# Autodesk Inventor assembly: centre wing
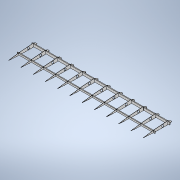
[picture p0: Inventor's stored thumbnail of the model, 180x180]
Saved by Autodesk Inventor 2021 (Build 250183000, 183)
## iProperties
Created: 2021-03-09
Part Number: centre wing
Document SubType Name: Assembly
Designer: Ferdinand Hubbard
Author: Ferdinand Hubbard
## Documents named in this file (4)
- C:\Users\Ferdinand Hubbard\Desktop\solarplane\cad\centre wing.iam
- C:\Users\Ferdinand Hubbard\Desktop\solarplane\cad\airfoil.ipt
- C:\Users\Ferdinand Hubbard\Desktop\solarplane\cad\centre back wood spar.ipt
- C:\Users\Ferdinand Hubbard\Desktop\solarplane\cad\centre front wood spar.ipt
## Components (14 placed, 3 different names)
1. airfoil:1 — Mate:1, Mate:2, Mate:9, Mate:60, Mate:61
2. centre back wood spar:1 — Mate:2, Mate:6, Mate:7, Mate:13, Mate:14, Mate:18, Mate:19, Mate:23, Mate:24, Mate:28, Mate:29, Mate:33, Mate:34, Mate:38, Mate:39, Mate:43, Mate:44, Mate:48, Mate:49, Mate:53, Mate:54, Mate:58, Mate:61, Mate:64
3. centre front wood spar:1 — Mate:1, Mate:5, Mate:8, Mate:11, Mate:12, Mate:16, Mate:17, Mate:21, Mate:22, Mate:26, Mate:27, Mate:31, Mate:32, Mate:36, Mate:37, Mate:41, Mate:42, Mate:46, Mate:47, Mate:51, Mate:52, Mate:56, Mate:60, Mate:63
4. airfoil:2 — Mate:5, Mate:6, Mate:7, Mate:8, Mate:9, Mate:10
5. airfoil:3 — Mate:10, Mate:11, Mate:12, Mate:13, Mate:14, Mate:15
6. airfoil:4 — Mate:15, Mate:16, Mate:17, Mate:18, Mate:19, Mate:20
7. airfoil:5 — Mate:20, Mate:21, Mate:22, Mate:23, Mate:24, Mate:25
8. airfoil:6 — Mate:25, Mate:26, Mate:27, Mate:28, Mate:29, Mate:30
9. airfoil:7 — Mate:30, Mate:31, Mate:32, Mate:33, Mate:34, Mate:35
10. airfoil:8 — Mate:35, Mate:36, Mate:37, Mate:38, Mate:39, Mate:40
11. airfoil:9 — Mate:40, Mate:41, Mate:42, Mate:43, Mate:44, Mate:45
12. airfoil:10 — Mate:45, Mate:46, Mate:47, Mate:48, Mate:49, Mate:50
13. airfoil:11 — Mate:50, Mate:51, Mate:52, Mate:53, Mate:54, Mate:55
14. airfoil:12 — Mate:55, Mate:56, Mate:58, Mate:63, Mate:64
## Relationships (59: Mate 59)
- Mate:1: airfoil:1 ↔ centre front wood spar:1
- Mate:2: airfoil:1 ↔ centre back wood spar:1
- Mate:5: centre front wood spar:1 ↔ airfoil:2
- Mate:6: centre back wood spar:1 ↔ airfoil:2
- Mate:7: centre back wood spar:1 ↔ airfoil:2
- Mate:8: centre front wood spar:1 ↔ airfoil:2
- Mate:9 (156.5 mm): airfoil:1 ↔ airfoil:2
- Mate:10 (156.5 mm): airfoil:2 ↔ airfoil:3
- Mate:11: centre front wood spar:1 ↔ airfoil:3
- Mate:12: centre front wood spar:1 ↔ airfoil:3
- Mate:13: centre back wood spar:1 ↔ airfoil:3
- Mate:14: centre back wood spar:1 ↔ airfoil:3
- Mate:15 (156.5 mm): airfoil:3 ↔ airfoil:4
- Mate:16: centre front wood spar:1 ↔ airfoil:4
- Mate:17: centre front wood spar:1 ↔ airfoil:4
- Mate:18: centre back wood spar:1 ↔ airfoil:4
- Mate:19: centre back wood spar:1 ↔ airfoil:4
- Mate:20 (156.5 mm): airfoil:4 ↔ airfoil:5
- Mate:21: centre front wood spar:1 ↔ airfoil:5
- Mate:22: centre front wood spar:1 ↔ airfoil:5
- Mate:23: centre back wood spar:1 ↔ airfoil:5
- Mate:24: centre back wood spar:1 ↔ airfoil:5
- Mate:25 (156.5 mm): airfoil:5 ↔ airfoil:6
- Mate:26: centre front wood spar:1 ↔ airfoil:6
- Mate:27: centre front wood spar:1 ↔ airfoil:6
- Mate:28: centre back wood spar:1 ↔ airfoil:6
- Mate:29: centre back wood spar:1 ↔ airfoil:6
- Mate:30 (156.5 mm): airfoil:6 ↔ airfoil:7
- Mate:31: centre front wood spar:1 ↔ airfoil:7
- Mate:32: centre front wood spar:1 ↔ airfoil:7
- Mate:33: centre back wood spar:1 ↔ airfoil:7
- Mate:34: centre back wood spar:1 ↔ airfoil:7
- Mate:35 (156.5 mm): airfoil:7 ↔ airfoil:8
- Mate:36: centre front wood spar:1 ↔ airfoil:8
- Mate:37: centre front wood spar:1 ↔ airfoil:8
- Mate:38: centre back wood spar:1 ↔ airfoil:8
- Mate:39: centre back wood spar:1 ↔ airfoil:8
- Mate:40 (156.5 mm): airfoil:8 ↔ airfoil:9
- Mate:41: centre front wood spar:1 ↔ airfoil:9
- Mate:42: centre front wood spar:1 ↔ airfoil:9
- Mate:43: centre back wood spar:1 ↔ airfoil:9
- Mate:44: centre back wood spar:1 ↔ airfoil:9
- Mate:45 (156.5 mm): airfoil:9 ↔ airfoil:10
- Mate:46: centre front wood spar:1 ↔ airfoil:10
- Mate:47: centre front wood spar:1 ↔ airfoil:10
- Mate:48: centre back wood spar:1 ↔ airfoil:10
- Mate:49: centre back wood spar:1 ↔ airfoil:10
- Mate:50 (156.5 mm): airfoil:10 ↔ airfoil:11
- Mate:51: centre front wood spar:1 ↔ airfoil:11
- Mate:52: centre front wood spar:1 ↔ airfoil:11
- Mate:53: centre back wood spar:1 ↔ airfoil:11
- Mate:54: centre back wood spar:1 ↔ airfoil:11
- Mate:55 (156.5 mm): airfoil:11 ↔ airfoil:12
- Mate:56: centre front wood spar:1 ↔ airfoil:12
- Mate:58: centre back wood spar:1 ↔ airfoil:12
- Mate:60: airfoil:1 ↔ centre front wood spar:1
- Mate:61: airfoil:1 ↔ centre back wood spar:1
- Mate:63 (20 mm): centre front wood spar:1 ↔ airfoil:12
- Mate:64 (20 mm): centre back wood spar:1 ↔ airfoil:12
